# Autodesk Inventor assembly: Picker Tool
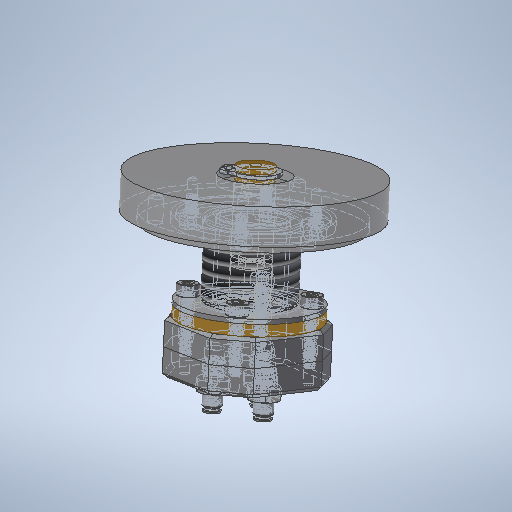
[picture p0: Inventor's stored thumbnail of the model, 512x512]
Saved by Autodesk Inventor 2025 (Build 290162000, 162)
## iProperties
Created: 2021-01-07
Part Number: Picker Tool
Document SubType Name: Assembly
Designer: caleb
Mass: 34.8876 g
Surface Area: 224.985 cm^2
Volume: 34.8876 cm^3
Density: 1 g/cm^3
Author: caleb
## Documents named in this file (7)
- C:\Users\cfang\Desktop\nebraska-silicon-lab\Hardware\ETL\Module Assembly\Picker Tool - V2\Picker Tool - V2.iam
- C:\Users\cfang\Desktop\nebraska-silicon-lab\Hardware\ETL\Module Assembly\Picker Tool\Picker Base.ipt
- C:\Users\cfang\Desktop\nebraska-silicon-lab\Hardware\ETL\Module Assembly\Picker Tool\Bellows Assembly.iam
- C:\Users\cfang\Desktop\nebraska-silicon-lab\Hardware\ETL\Module Assembly\Picker Tool\Spool Assembly.iam
- C:\Users\cfang\Desktop\nebraska-silicon-lab\Hardware\ETL\Module Assembly\Picker Tool - V2\Platform Assembly - V2.iam
- C:\Users\cfang\Desktop\nebraska-silicon-lab\Hardware\ETL\Module Assembly\Picker Tool - V2\91290A099_Alloy Steel Socket Head Screw\91290A099_Alloy Steel Socket Head Screw.ipt
- C:\Users\cfang\Desktop\nebraska-silicon-lab\Hardware\ETL\Module Assembly\Picker Tool - V2\91290A104_Alloy Steel Socket Head Screw\91290A104_Alloy Steel Socket Head Screw.ipt
## Components (12 placed, 6 different names)
1. Picker Base:1 — Insert:13, Insert:14
2. Bellows Assembly:1 [sub-assembly] — Insert:13, Insert:14, Mate:1, Insert:15, Insert:16, Insert:19, Insert:20, Insert:21, Insert:22, Insert:23, Insert:24, Insert:25, Insert:26
3. Platform Assembly - V2:1 [sub-assembly] — Insert:17, Insert:18
4. Spool Assembly:1 [sub-assembly] — Mate:1, Insert:15, Insert:16, Insert:17, Insert:18
5. 91290A099_Alloy Steel Socket Head Screw:1 — Insert:19
6. 91290A099_Alloy Steel Socket Head Screw:2 — Insert:20
7. 91290A099_Alloy Steel Socket Head Screw:3 — Insert:21
8. 91290A099_Alloy Steel Socket Head Screw:4 — Insert:22
9. 91290A104_Alloy Steel Socket Head Screw:1 — Insert:25
10. 91290A104_Alloy Steel Socket Head Screw:2 — Insert:26
11. 91290A104_Alloy Steel Socket Head Screw:3 — Insert:24
12. 91290A104_Alloy Steel Socket Head Screw:4 — Insert:23
## Relationships (15: Insert 14, Mate 1)
- Insert:13: Picker Base:1 ↔ Bellows Assembly:1
- Insert:14: Picker Base:1 ↔ Bellows Assembly:1
- Mate:1: Bellows Assembly:1 ↔ Spool Assembly:1
- Insert:15: Bellows Assembly:1 ↔ Spool Assembly:1
- Insert:16: Bellows Assembly:1 ↔ Spool Assembly:1
- Insert:17: Platform Assembly - V2:1 ↔ Spool Assembly:1
- Insert:18: Platform Assembly - V2:1 ↔ Spool Assembly:1
- Insert:19: Bellows Assembly:1 ↔ 91290A099_Alloy Steel Socket Head Screw:1
- Insert:20: Bellows Assembly:1 ↔ 91290A099_Alloy Steel Socket Head Screw:2
- Insert:21: Bellows Assembly:1 ↔ 91290A099_Alloy Steel Socket Head Screw:3
- Insert:22: Bellows Assembly:1 ↔ 91290A099_Alloy Steel Socket Head Screw:4
- Insert:23: Bellows Assembly:1 ↔ 91290A104_Alloy Steel Socket Head Screw:4
- Insert:24: Bellows Assembly:1 ↔ 91290A104_Alloy Steel Socket Head Screw:3
- Insert:25: Bellows Assembly:1 ↔ 91290A104_Alloy Steel Socket Head Screw:1
- Insert:26: Bellows Assembly:1 ↔ 91290A104_Alloy Steel Socket Head Screw:2
